# Autodesk Inventor assembly: Gauge Controller
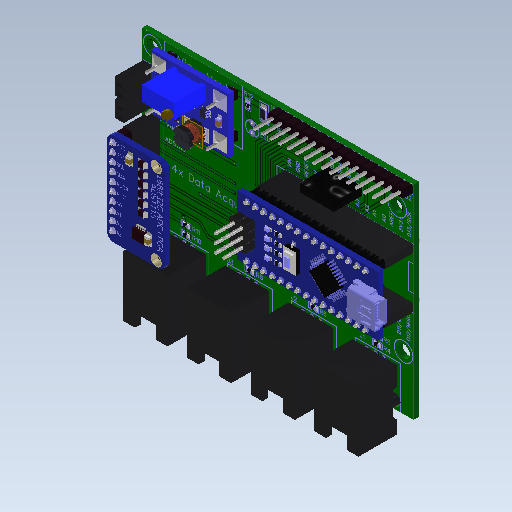
[picture p0: Inventor's stored thumbnail of the model, 512x512]
Saved by Autodesk Inventor 2020 (Build 240168000, 168)
## iProperties
Created: 2019-11-12
Part Number: Gauge Controller
Document SubType Name: Assembly
Designer: Alex
Author: Alex
## Documents named in this file (14)
- C:\Users\amsmi\Google Drive\Pirani Gauge\Pirani Gauge Modeling\Data Acquisition\Gauge Controller.iam
- C:\Users\amsmi\Google Drive\Pirani Gauge\Pirani Gauge Modeling\Data Acquisition\Boost Converter.iam
- C:\Users\amsmi\Google Drive\Pirani Gauge\Pirani Gauge Modeling\Data Acquisition\PCB.ipt
- C:\Users\amsmi\Google Drive\Pirani Gauge\Pirani Gauge Modeling\Data Acquisition\ADS1115.ipt
- C:\Users\amsmi\Google Drive\Pirani Gauge\Pirani Gauge Modeling\Data Acquisition\RJ12 - 90deg.ipt
- C:\Users\amsmi\Google Drive\Pirani Gauge\Pirani Gauge Modeling\Data Acquisition\16 pin header.ipt
- C:\Users\amsmi\Google Drive\Pirani Gauge\Pirani Gauge Modeling\Data Acquisition\15 female pin.ipt
- C:\Users\amsmi\Google Drive\Pirani Gauge\Pirani Gauge Modeling\Data Acquisition\2  female pin.ipt
- C:\Users\amsmi\Google Drive\Pirani Gauge\Pirani Gauge Modeling\Data Acquisition\4  female pin.ipt
- C:\Users\amsmi\Google Drive\Pirani Gauge\Pirani Gauge Modeling\Data Acquisition\10 female pin.ipt
- C:\Users\amsmi\Google Drive\Pirani Gauge\Pirani Gauge Modeling\Data Acquisition\10 pin header.ipt
- C:\Users\amsmi\Google Drive\Pirani Gauge\Pirani Gauge Modeling\Data Acquisition\Arduino Nano - Soldered.iam
- C:\Users\amsmi\Google Drive\Pirani Gauge\Pirani Gauge Modeling\Data Acquisition\Black 0603 - Soldered.ipt
- C:\Users\amsmi\Google Drive\Pirani Gauge\Pirani Gauge Modeling\Data Acquisition\Black 1206 - Soldered.ipt
## Components (32 placed, 13 different names)
1. Boost Converter:1 [sub-assembly] — Mate:4, Angle:1, Mate:31
2. PCB:1 — Mate:1, Mate:2, Mate:3, Mate:4, Angle:1, Mate:5, Mate:6, Mate:7, Mate:8, Mate:9, Angle:2, Mate:13, Mate:14, Mate:16, Angle:3, Mate:18, Mate:19, Mate:20, Mate:21, Mate:22, Mate:23, Mate:24, Mate:25, Angle:4, Mate:27, Mate:28, Angle:6, Mate:29, Mate:30, Angle:7, Mate:31
3. ADS1115:1 — Mate:11, Mate:12
4. 16 pin header:1 — Mate:7
5. 15 female pin:1 — Mate:5, Flush:7, Flush:8
6. 15 female pin:2 — Mate:6, Mate:17, Flush:5, Flush:6
7. 2  female pin:1 — Flush:3, Flush:4, Mate:16, Angle:3
8. 2  female pin:2 — Flush:3, Flush:4
9. 4  female pin:1 — Mate:8
10. 10 female pin:1 — Mate:9, Mate:10, Flush:1, Flush:2, Angle:2
11. 10 pin header:1 — Mate:10, Flush:1, Flush:2, Mate:11, Mate:12
12. Arduino Nano - Soldered:1 [sub-assembly] — Mate:17, Flush:5, Flush:6, Flush:7, Flush:8
13. Black 0603 - Soldered:2 — Mate:21
14. Black 0603 - Soldered:9 — Mate:19
15. Black 0603 - Soldered:10 — Mate:20
16. Black 0603 - Soldered:11 — Mate:22
17. Black 0603 - Soldered:12 — Mate:23
18. Black 0603 - Soldered:13 — Mate:24
19. Black 0603 - Soldered:14 — Mate:25, Angle:4
20. Black 0603 - Soldered:15 — Mate:28, Angle:6
21. Black 0603 - Soldered:16 — Mate:27
22. Black 0603 - Soldered:17 — Mate:29
23. Black 1206 - Soldered:1 — Mate:30, Angle:7
24. RJ12 - 90deg:1 — Mate:13, Mate:14
25. RJ12 - 90deg:2
26. RJ12 - 90deg:3
27. RJ12 - 90deg:4
28. Black 0603 - Soldered:1 — Mate:18
29. Black 0603 - Soldered:5
30. Black 0603 - Soldered:6
31. Black 0603 - Soldered:7
32. Black 0603 - Soldered:8
## Component patterns: (4 elements, first: RJ12 - 90deg:1), (8 elements, first: Black 0603 - Soldered:1)
## Relationships (43: Mate 29, Flush 8, Angle 6)
- Mate:1: PCB:1
- Mate:2: PCB:1
- Mate:3: PCB:1
- Mate:4: Boost Converter:1 ↔ PCB:1
- Angle:1 (0 deg): Boost Converter:1 ↔ PCB:1
- Mate:5: PCB:1 ↔ 15 female pin:1
- Mate:6: PCB:1 ↔ 15 female pin:2
- Mate:7: PCB:1 ↔ 16 pin header:1
- Mate:8: PCB:1 ↔ 4  female pin:1
- Mate:9: PCB:1 ↔ 10 female pin:1
- Mate:10: 10 female pin:1 ↔ 10 pin header:1
- Flush:1: 10 female pin:1 ↔ 10 pin header:1
- Flush:2: 10 female pin:1 ↔ 10 pin header:1
- Mate:11: ADS1115:1 ↔ 10 pin header:1
- Mate:12: ADS1115:1 ↔ 10 pin header:1
- Angle:2 (0 deg): PCB:1 ↔ 10 female pin:1
- Mate:13: PCB:1 ↔ RJ12 - 90deg:1
- Mate:14: PCB:1 ↔ RJ12 - 90deg:1
- Flush:3: 2  female pin:1 ↔ 2  female pin:2
- Flush:4: 2  female pin:1 ↔ 2  female pin:2
- Mate:16: PCB:1 ↔ 2  female pin:1
- Angle:3 (0 deg): PCB:1 ↔ 2  female pin:1
- Mate:17: 15 female pin:2 ↔ Arduino Nano - Soldered:1
- Flush:5: 15 female pin:2 ↔ Arduino Nano - Soldered:1
- Flush:6: 15 female pin:2 ↔ Arduino Nano - Soldered:1
- Flush:7: 15 female pin:1 ↔ Arduino Nano - Soldered:1
- Flush:8: 15 female pin:1 ↔ Arduino Nano - Soldered:1
- Mate:18: PCB:1 ↔ Black 0603 - Soldered:1
- Mate:19: PCB:1 ↔ Black 0603 - Soldered:9
- Mate:20: PCB:1 ↔ Black 0603 - Soldered:10
- Mate:21: PCB:1 ↔ Black 0603 - Soldered:2
- Mate:22: PCB:1 ↔ Black 0603 - Soldered:11
- Mate:23: PCB:1 ↔ Black 0603 - Soldered:12
- Mate:24: PCB:1 ↔ Black 0603 - Soldered:13
- Mate:25: PCB:1 ↔ Black 0603 - Soldered:14
- Angle:4 (0 deg): PCB:1 ↔ Black 0603 - Soldered:14
- Mate:27: PCB:1 ↔ Black 0603 - Soldered:16
- Mate:28: PCB:1 ↔ Black 0603 - Soldered:15
- Angle:6 (0 deg): PCB:1 ↔ Black 0603 - Soldered:15
- Mate:29: PCB:1 ↔ Black 0603 - Soldered:17
- Mate:30: PCB:1 ↔ Black 1206 - Soldered:1
- Angle:7 (0 deg): PCB:1 ↔ Black 1206 - Soldered:1
- Mate:31: Boost Converter:1 ↔ PCB:1
